# Autodesk Inventor assembly: wheel with drive motor floor
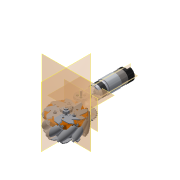
[picture p0: Inventor's stored thumbnail of the model, 180x180]
Saved by Autodesk Inventor 2018 (Build 220112000, 112)
## iProperties
Created: 2019-10-04
Part Number: wheel with drive motor floor
Document SubType Name: Assembly
Designer: ball
Author: ball
## Documents named in this file (3)
- C:\FTC\FTC8863CAD\2019 Robot\Mecanum Drive Train\wheel with drive motor top.iam
- C:\FTC\FTC8863CAD\2019 Robot\Mecanum Drive Train\motor with bevil gear and sprocket.iam
- C:\FTC\FTC8863CAD\2019 Robot\Mecanum Drive Train\wheel with sprocket.iam
## Components (2 placed, 2 different names)
1. motor with bevil gear and sprocket:1 [sub-assembly] — Flush:2, Flush:3, Flush:4
2. wheel with sprocket:1 [sub-assembly] — Flush:2, Flush:3, Flush:4
## Relationships (3: Flush 3)
- Flush:2 (-33.02 mm): motor with bevil gear and sprocket:1 ↔ wheel with sprocket:1
- Flush:3: motor with bevil gear and sprocket:1 ↔ wheel with sprocket:1
- Flush:4 (76.2 mm): motor with bevil gear and sprocket:1 ↔ wheel with sprocket:1
